# Autodesk Inventor assembly: pałka
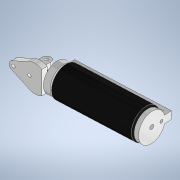
[picture p0: Inventor's stored thumbnail of the model, 180x180]
Saved by Autodesk Inventor 2022.3 (Build 263350000, 350)
## iProperties
Created: 2022-11-16
Part Number: pałka
Document SubType Name: Assembly
Designer: komputer
Author: komputer
## Documents named in this file (7)
- C:\Users\komputer\pałka.iam
- C:\Users\komputer\Desktop\MicroGearmotor v3.ipt
- C:\Users\komputer\Part6.ipt
- C:\Users\komputer\Downloads\Motor Bracket.ipt
- C:\Users\komputer\Part9.ipt
- C:\Users\komputer\Part10.ipt
- C:\Users\komputer\Part11.ipt
## Components (6 placed, 6 different names)
1. MicroGearmotor v3:1 — Flush:1, Flush:2, Mate:1, Mate:2, Flush:3
2. Part6:1 — Flush:1
3. Motor Bracket:1 — Flush:2, Mate:1, Mate:2, Flush:4, Flush:5, Mate:3, Mate:4
4. Part9:1 — Flush:3
5. Part11:1 — Flush:4, Flush:5
6. Part10:1 — Mate:3, Mate:4
## Relationships (9: Flush 5, Mate 4)
- Flush:1: MicroGearmotor v3:1 ↔ Part6:1
- Flush:2: MicroGearmotor v3:1 ↔ Motor Bracket:1
- Mate:1: MicroGearmotor v3:1 ↔ Motor Bracket:1
- Mate:2: MicroGearmotor v3:1 ↔ Motor Bracket:1
- Flush:3: MicroGearmotor v3:1 ↔ Part9:1
- Flush:4: Motor Bracket:1 ↔ Part11:1
- Flush:5: Motor Bracket:1 ↔ Part11:1
- Mate:3: Motor Bracket:1 ↔ Part10:1
- Mate:4: Motor Bracket:1 ↔ Part10:1
